# Autodesk Inventor assembly: Assembly2
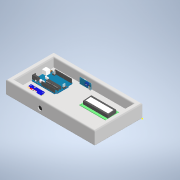
[picture p0: Inventor's stored thumbnail of the model, 180x180]
Saved by Autodesk Inventor 2022 (Build 260153000, 153)
## iProperties
Created: 2022-05-06
Part Number: Assembly2
Document SubType Name: Assembly
Designer: Asus
Author: Asus
## Documents named in this file (7)
- E:\Engineering mac. Project\Assembly2.iam
- E:\Engineering mac. Project\box final.ipt
- E:\Engineering mac. Project\ARDUINO.ipt
- E:\Engineering mac. Project\GAS SENSOR.ipt
- E:\Engineering mac. Project\LCD.ipt
- E:\Engineering mac. Project\SIM.ipt
- E:\Engineering mac. Project\Buzzer.ipt
## Components (6 placed, 6 different names)
1. box final:1 — Insert:1
2. ARDUINO:1 — Insert:1
3. GAS SENSOR:1
4. LCD:1
5. SIM:1
6. Buzzer:1
## Relationships (1: Insert 1)
- Insert:1: box final:1 ↔ ARDUINO:1
